# Autodesk Inventor assembly: EnsamblajeDodecaedro_V3_soportes
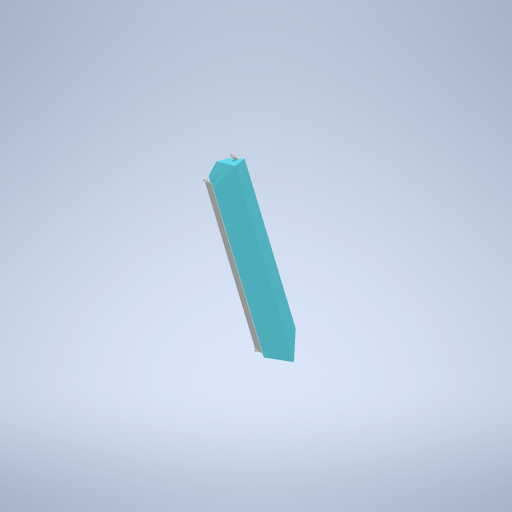
[picture p0: Inventor's stored thumbnail of the model, 512x512]
Saved by Autodesk Inventor 2024 (Build 280153000, 153)
## iProperties
Created: 2023-08-17
Part Number: EnsamblajeDodecaedro_V3_soportes
Document SubType Name: Assembly
Designer: sergi
Author: sergi
## Documents named in this file (3)
- C:\Users\sergi\OneDrive\Escritorio\Piso\Dodecaedro\EnsamblajeDodecaedro_V3_soportes.iam
- C:\Users\sergi\OneDrive\Escritorio\Piso\Dodecaedro\Perfil_V3.ipt
- C:\Users\sergi\OneDrive\Escritorio\Piso\Dodecaedro\Soportes.ipt
## Components (2 placed, 2 different names)
1. Perfil_V3:1 — Coincidencia:1, Nivelación:1, Nivelación:2, Coincidencia:2, Coincidencia:3
2. Soportes:1 — Nivelación:1, Nivelación:2, Coincidencia:2, Coincidencia:3
## Relationships (5: Mate 3, Flush 2)
- Coincidencia:1 [Mate]: Perfil_V3:1
- Nivelación:1 [Flush]: Perfil_V3:1 ↔ Soportes:1
- Nivelación:2 [Flush]: Perfil_V3:1 ↔ Soportes:1
- Coincidencia:2 [Mate]: Perfil_V3:1 ↔ Soportes:1
- Coincidencia:3 [Mate]: Perfil_V3:1 ↔ Soportes:1
